# Autodesk Inventor assembly: compliant wheel 2 in + motor adapter
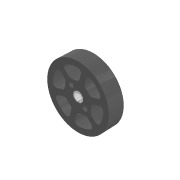
[picture p0: Inventor's stored thumbnail of the model, 180x180]
Saved by Autodesk Inventor 2020 (Build 240168000, 168)
## iProperties
Created: 2019-11-08
Part Number: compliant wheel 2 in + motor adapter
Document SubType Name: Assembly
Designer: ball
Author: ball
## Documents named in this file (3)
- C:\FTC\FTC8863CAD\2019 Robot\Collection\compliant wheel 2 in + motor adapter.iam
- C:\FTC\FTC8863CAD\Andymark\am-3572 2IN 8mm Compliant Wheel REV2.ipt
- C:\FTC\FTC8863CAD\2019 Robot\Generic Parts\clamping hub 6mm to 8mm hub.ipt
## Components (2 placed, 2 different names)
1. am-3572 2IN 8mm Compliant Wheel REV2:1 — Mate:1, Mate:2, Mate:3
2. clamping hub 6mm to 8mm hub:1 — Mate:1, Mate:2, Mate:3
## Relationships (3: Mate 3)
- Mate:1: am-3572 2IN 8mm Compliant Wheel REV2:1 ↔ clamping hub 6mm to 8mm hub:1
- Mate:2: am-3572 2IN 8mm Compliant Wheel REV2:1 ↔ clamping hub 6mm to 8mm hub:1
- Mate:3: am-3572 2IN 8mm Compliant Wheel REV2:1 ↔ clamping hub 6mm to 8mm hub:1
